# Autodesk Inventor assembly: !Conveyer
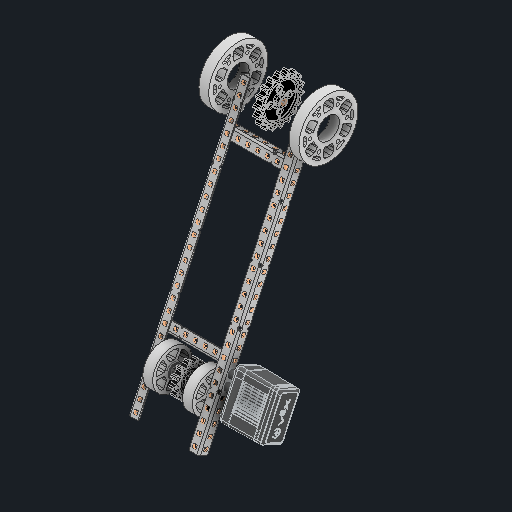
[picture p0: Inventor's stored thumbnail of the model, 512x512]
Saved by Autodesk Inventor 2025 (Build 290162000, 162)
## iProperties
Created: 2024-12-25
Part Number: !Conveyer
Document SubType Name: Assembly
Designer: Averey Ku
Author: Averey Ku
## Documents named in this file (7)
- D:\VEX\High Stakes\CAD\V4\Conveyer\!Conveyer.iam
- D:\VEX\High Stakes\CAD\V4\Conveyer\Structure.iam
- D:\VEX\High Stakes\CAD\V4\Conveyer\Bottom Roller.iam
- D:\VEX\High Stakes\CAD\ROBOPROS-CAD-Inventor\Motion\Sprockets\9P Sprocket\9P 18T Sprocket, No Insert.iam
- D:\VEX\High Stakes\CAD\ROBOPROS-CAD-Inventor\Motion\Sprockets\9P Sprocket.iam
- D:\VEX\High Stakes\CAD\ROBOPROS-CAD-Inventor\Motion\Wheels\Flex Wheels\3.000 Flex Wheel\3.000 30A .500.ipt
- D:\VEX\High Stakes\CAD\ROBOPROS-CAD-Inventor\Motion\Wheels\Flex Wheels\3.000 Flex Wheel.ipt
## Components (5 placed, 4 different names)
1. Structure:1 [sub-assembly] — Insert:1, Mate:1, Insert:2, Insert:3
2. Bottom Roller:1 [sub-assembly] — Insert:1, Flush:1
3. 9P 18T Sprocket, No Insert:1 [sub-assembly] — Mate:1, Flush:1
4. 3.000 30A .500:1 — Insert:3
5. 3.000 30A .500:2 — Insert:2
## Relationships (5: Insert 3, Mate 1, Flush 1)
- Insert:1 (9.525 mm): Structure:1 ↔ Bottom Roller:1
- Mate:1: Structure:1 ↔ 9P 18T Sprocket, No Insert:1
- Flush:1: Bottom Roller:1 ↔ 9P 18T Sprocket, No Insert:1
- Insert:2 (6.35 mm): Structure:1 ↔ 3.000 30A .500:2
- Insert:3 (6.35 mm): Structure:1 ↔ 3.000 30A .500:1
